# Autodesk Inventor assembly: ControlBoxAssembly
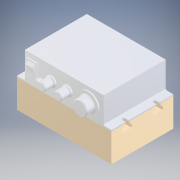
[picture p0: Inventor's stored thumbnail of the model, 180x180]
Saved by Autodesk Inventor 2017 (Build 210142000, 142)
## iProperties
Created: 2018-08-13
Part Number: ControlBoxAssembly
Document SubType Name: Assembly
Designer: Jake
Author: Jake
## Documents named in this file (4)
- C:\Users\Jake\git\CAD-Projects\StereoCabinet\ControlBoxAssembly.iam
- C:\Users\Jake\git\CAD-Projects\StereoCabinet\controlBox.ipt
- C:\Users\Jake\git\CAD-Projects\StereoCabinet\AmpLP2020A.ipt
- C:\Users\Jake\git\CAD-Projects\parts\RaspberryPi3B+.ipt
## Components (3 placed, 3 different names)
1. controlBox:1 — Mate:1, Flush:1, Flush:2, Mate:2, Mate:3, Mate:4
2. AmpLP2020A:1 — Mate:1, Flush:1, Flush:2
3. RaspberryPi3B+:1 — Mate:2, Mate:3, Mate:4
## Relationships (6: Mate 4, Flush 2)
- Mate:1: controlBox:1 ↔ AmpLP2020A:1
- Flush:1: controlBox:1 ↔ AmpLP2020A:1
- Flush:2: controlBox:1 ↔ AmpLP2020A:1
- Mate:2: controlBox:1 ↔ RaspberryPi3B+:1
- Mate:3: controlBox:1 ↔ RaspberryPi3B+:1
- Mate:4: controlBox:1 ↔ RaspberryPi3B+:1
